# Autodesk Inventor assembly: ShockAbsorber
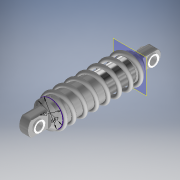
[picture p0: Inventor's stored thumbnail of the model, 180x180]
Saved by Autodesk Inventor 2016 (Build 200138000, 138)
## iProperties
Created: 2013-09-01
Part Number: ShockAbsorber
Document SubType Name: Assembly
Designer: Arto
Author: Arto
## Documents named in this file (6)
- C:\Users\Yann\Documents\GitHub\BIKAIR_CAD\Source\Rear_Train\Suspension\ShockAbsorber.iam
- C:\Users\Yann\Documents\GitHub\BIKAIR_CAD\Source\Rear_train\Suspension\Spring_shockabsorber.ipt
- C:\Users\Yann\Documents\GitHub\BIKAIR_CAD\Source\Rear_train\Suspension\Base.ipt
- C:\Users\Yann\Documents\GitHub\BIKAIR_CAD\Source\Rear_train\Suspension\PistonRod.ipt
- C:\Users\Yann\Documents\GitHub\BIKAIR_CAD\Source\Rear_train\Suspension\Top.ipt
- C:\Users\Yann\Documents\GitHub\BIKAIR_CAD\Source\Rear_train\Suspension\Holkki.ipt
## Components (6 placed, 5 different names)
1. Spring_shockabsorber:1
2. Base:1 — Flush:1, Insert:1
3. PistonRod:1 — Flush:3
4. Top:1 — Flush:4, Flush:5
5. Holkki:1 — Flush:5
6. Holkki:2 — Insert:1
## Relationships (6: Flush 5, Insert 1)
- Flush:1: Base:1
- Flush:2 (210 mm)
- Flush:3: PistonRod:1
- Flush:4: Top:1
- Flush:5: Top:1 ↔ Holkki:1
- Insert:1: Base:1 ↔ Holkki:2
